# Autodesk Inventor assembly: Zespół3
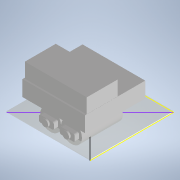
[picture p0: Inventor's stored thumbnail of the model, 180x180]
Saved by Autodesk Inventor 2020 (Build 240168000, 168)
## iProperties
Created: 2019-06-28
Part Number: Zespół3
Document SubType Name: Assembly
Designer: atmat
Author: atmat
## Documents named in this file (5)
- C:\Users\atmat\Documents\1.Projects\1.Roboty\1.Rainbow\1.Reincarnation\Czesci\Ver 2\Zespół3.iam
- C:\Users\atmat\Documents\1.Projects\1.Roboty\1.Rainbow\1.Reincarnation\Czesci\Ver 2\Silnik_SKUA.ipt
- C:\Users\atmat\Documents\1.Projects\1.Roboty\1.Rainbow\1.Reincarnation\Czesci\Ver 2\Platworma_10x10.ipt
- C:\Users\atmat\Documents\1.Projects\1.Roboty\1.Rainbow\1.Reincarnation\Czesci\Ver 2\Bateria_22V2.ipt
- C:\Users\atmat\Documents\1.Projects\1.Roboty\1.Rainbow\1.Reincarnation\Czesci\Ver 2\Bateria_22V2_Rozlozona.ipt
## Components (5 placed, 4 different names)
1. Silnik_SKUA:1 — Równoległe:1, Równoległe:2, Równoległe:3, Zestawiające:2
2. Silnik_SKUA:2 — Równoległe:1, Równoległe:2, Równoległe:3, Zestawiające:1
3. Platworma_10x10:1 — Zestawiające:1
4. Bateria_22V2:1 — Zestawiające:2, Równoległe:4
5. Bateria_22V2_Rozlozona:1 — Równoległe:4
## Relationships (6: Flush 4, Mate 2)
- Równoległe:1 [Flush]: Silnik_SKUA:1 ↔ Silnik_SKUA:2
- Równoległe:2 [Flush] (25 mm): Silnik_SKUA:1 ↔ Silnik_SKUA:2
- Równoległe:3 [Flush]: Silnik_SKUA:1 ↔ Silnik_SKUA:2
- Zestawiające:1 [Mate]: Silnik_SKUA:2 ↔ Platworma_10x10:1
- Zestawiające:2 [Mate] (12.5 mm): Silnik_SKUA:1 ↔ Bateria_22V2:1
- Równoległe:4 [Flush]: Bateria_22V2:1 ↔ Bateria_22V2_Rozlozona:1
